# Autodesk Inventor assembly: PostBaseJigs
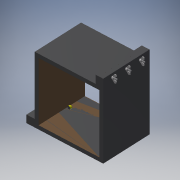
[picture p0: Inventor's stored thumbnail of the model, 180x180]
Saved by Autodesk Inventor 2016 (Build 200138000, 138)
## iProperties
Created: 2015-06-07
Part Number: PostBaseJigs
Document SubType Name: Assembly
Designer: krosie
Author: krosie
## Documents named in this file (5)
- C:\Users\krosie\Google Drive\HERA\hera-cad\jigs\PostBaseJigs.iam
- C:\Users\krosie\Google Drive\HERA\hera-cad\jigs\ConcreteFormwork.ipt
- C:\Users\krosie\Google Drive\HERA\hera-cad\jigs\ConcreteFormwork2.ipt
- C:\Users\krosie\Documents\Inventor\Content Center Files\R2016\en-US\JIS B 1185 T 1\JIS B 1185 - M8.ipt
- C:\Users\krosie\Documents\Inventor\Content Center Files\R2016\en-US\AS 1111\AS 1111 - M8 x 60.ipt
## Components (14 placed, 4 different names)
1. ConcreteFormwork1:1 — Mate:1, Mate:2, Mate:3, Mate:4, Mate:7, Mate:22, Mate:24, Mate:26, Mate:28, Mate:30, Angle:1, Angle:2, Angle:3, Angle:4, Angle:5, Angle:6
2. ConcreteFormwork2:1 — Mate:1, Mate:2, Mate:3, Mate:4
3. AS 1111 - Metric M8 x 60:1
4. JIS B 1185 Type 1 - Metric M8:7 — Mate:7, Angle:1
5. AS 1111 - Metric M8 x 60:2
6. AS 1111 - Metric M8 x 60:3
7. AS 1111 - Metric M8 x 60:4
8. AS 1111 - Metric M8 x 60:5
9. AS 1111 - Metric M8 x 60:6
10. JIS B 1185 Type 1 - Metric M8:8 — Mate:22, Angle:2
11. JIS B 1185 Type 1 - Metric M8:9 — Mate:24, Angle:3
12. JIS B 1185 Type 1 - Metric M8:10 — Mate:26, Angle:4
13. JIS B 1185 Type 1 - Metric M8:11 — Mate:28, Angle:5
14. JIS B 1185 Type 1 - Metric M8:12 — Mate:30, Angle:6
## Relationships (34: Mate 28, Angle 6)
- Mate:1: ConcreteFormwork1:1 ↔ ConcreteFormwork2:1
- Mate:2: ConcreteFormwork1:1 ↔ ConcreteFormwork2:1
- Mate:3: ConcreteFormwork1:1 ↔ ConcreteFormwork2:1
- Mate:4: ConcreteFormwork1:1 ↔ ConcreteFormwork2:1
- [Mate]: ConcreteFormwork2:1 ↔ AS 1111 - Metric M8 x 60:1
- [Mate]: AS 1111 - Metric M8 x 60:1 ↔ JIS B 1185 Type 1 - Metric M8:7
- Mate:7: ConcreteFormwork1:1 ↔ JIS B 1185 Type 1 - Metric M8:7
- [Mate]: ConcreteFormwork2:1 ↔ AS 1111 - Metric M8 x 60:1
- [Mate]: ConcreteFormwork2:1 ↔ AS 1111 - Metric M8 x 60:2
- [Mate]: ConcreteFormwork2:1 ↔ AS 1111 - Metric M8 x 60:2
- [Mate]: ConcreteFormwork2:1 ↔ AS 1111 - Metric M8 x 60:3
- [Mate]: ConcreteFormwork2:1 ↔ AS 1111 - Metric M8 x 60:3
- [Mate]: ConcreteFormwork2:1 ↔ AS 1111 - Metric M8 x 60:4
- [Mate]: ConcreteFormwork2:1 ↔ AS 1111 - Metric M8 x 60:4
- [Mate]: ConcreteFormwork2:1 ↔ AS 1111 - Metric M8 x 60:5
- [Mate]: ConcreteFormwork2:1 ↔ AS 1111 - Metric M8 x 60:5
- [Mate]: ConcreteFormwork2:1 ↔ AS 1111 - Metric M8 x 60:6
- [Mate]: ConcreteFormwork2:1 ↔ AS 1111 - Metric M8 x 60:6
- [Mate]: AS 1111 - Metric M8 x 60:2 ↔ JIS B 1185 Type 1 - Metric M8:8
- Mate:22: ConcreteFormwork1:1 ↔ JIS B 1185 Type 1 - Metric M8:8
- [Mate]: AS 1111 - Metric M8 x 60:3 ↔ JIS B 1185 Type 1 - Metric M8:9
- Mate:24: ConcreteFormwork1:1 ↔ JIS B 1185 Type 1 - Metric M8:9
- [Mate]: AS 1111 - Metric M8 x 60:4 ↔ JIS B 1185 Type 1 - Metric M8:10
- Mate:26: ConcreteFormwork1:1 ↔ JIS B 1185 Type 1 - Metric M8:10
- [Mate]: AS 1111 - Metric M8 x 60:6 ↔ JIS B 1185 Type 1 - Metric M8:11
- Mate:28: ConcreteFormwork1:1 ↔ JIS B 1185 Type 1 - Metric M8:11
- [Mate]: AS 1111 - Metric M8 x 60:5 ↔ JIS B 1185 Type 1 - Metric M8:12
- Mate:30: ConcreteFormwork1:1 ↔ JIS B 1185 Type 1 - Metric M8:12
- Angle:1 (0 deg): ConcreteFormwork1:1 ↔ JIS B 1185 Type 1 - Metric M8:7
- Angle:2 (0 deg): ConcreteFormwork1:1 ↔ JIS B 1185 Type 1 - Metric M8:8
- Angle:3 (0 deg): ConcreteFormwork1:1 ↔ JIS B 1185 Type 1 - Metric M8:9
- Angle:4 (0 deg): ConcreteFormwork1:1 ↔ JIS B 1185 Type 1 - Metric M8:10
- Angle:5 (0 deg): ConcreteFormwork1:1 ↔ JIS B 1185 Type 1 - Metric M8:11
- Angle:6 (0 deg): ConcreteFormwork1:1 ↔ JIS B 1185 Type 1 - Metric M8:12
